# Autodesk Inventor assembly: Elevator Latch Assembly
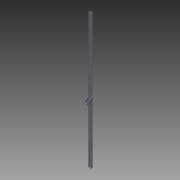
[picture p0: Inventor's stored thumbnail of the model, 180x180]
Saved by Autodesk Inventor 2015 (Build 190159000, 159)
## iProperties
Created: 2015-01-31
Part Number: Elevator Latch Assembly
Document SubType Name: Assembly
Designer: chapale16
Author: chapale16
## Documents named in this file (4)
- \\lhssvr02\Homedirs\Robotics Club\CAD Model 2015\Elevator Latch Assembly.iam
- \\lhssvr02\Homedirs\Robotics Club\CAD Model 2015\Parts Folder\Stock\c hannel.ipt
- \\lhssvr02\Homedirs\Robotics Club\CAD Model 2015\Box Beam Drive Base\Elevator Latch.ipt
- \\lhssvr02\Homedirs\Robotics Club\CAD Model 2015\Pin.ipt
## Components (6 placed, 3 different names)
1. c hannel:1 — Mate:3, Mate:4, Mate:5, Flush:3, Mate:8
2. Elevator Latch:1 — Mate:1, Mate:2, Mate:3, Mate:4, Mate:6, Flush:2, Mate:7
3. Elevator Latch:2 — Mate:1, Mate:2, Mate:5, Flush:1
4. Pin:1 — Mate:6, Flush:1
5. Pin:2 — Flush:2, Mate:7
6. Pin:3 — Flush:3, Mate:8
## Relationships (11: Mate 8, Flush 3)
- Mate:1: Elevator Latch:1 ↔ Elevator Latch:2
- Mate:2: Elevator Latch:1 ↔ Elevator Latch:2
- Mate:3 (2.54 mm): c hannel:1 ↔ Elevator Latch:1
- Mate:4: c hannel:1 ↔ Elevator Latch:1
- Mate:5 (2.54 mm): c hannel:1 ↔ Elevator Latch:2
- Mate:6: Elevator Latch:1 ↔ Pin:1
- Flush:1 (3.175 mm): Elevator Latch:2 ↔ Pin:1
- Flush:2 (-6.35 mm): Elevator Latch:1 ↔ Pin:2
- Mate:7: Elevator Latch:1 ↔ Pin:2
- Flush:3 (-3.175 mm): c hannel:1 ↔ Pin:3
- Mate:8: c hannel:1 ↔ Pin:3
